# Autodesk Inventor assembly: Motor_25GA370-226x1-6V-21RPM
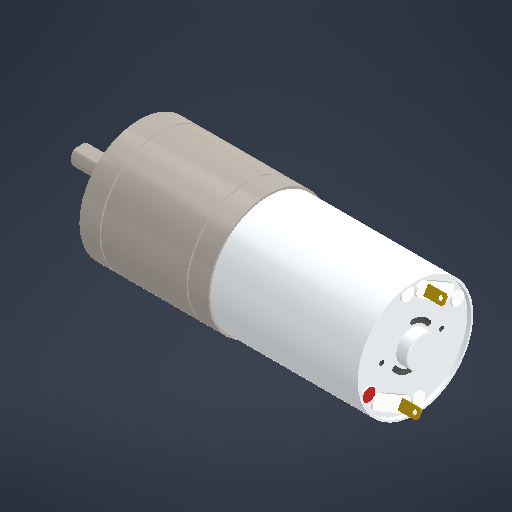
[picture p0: Inventor's stored thumbnail of the model, 512x512]
Saved by Autodesk Inventor 2026.1 (Build 301233000, 233)
## iProperties
Created: 2023-10-13
Part Number: Motor_25GA370-226x1-6V-21RPM
Description: STEP AP214
Document SubType Name: Assembly
Designer: pc
Sending System: SolidWorks 2022
Preprocessor: SwSTEP 2.0
Title: Motor_25GA370-226x1-6V-21RPM.STEP
Author: Wurs
Revision Number: ANY
## Documents named in this file (3)
- D:\momen\Eng.-ASU\Senior1\MCT Sys design\design\old design\Motor_25GA370-226x1-6V-21RPM.iam
- D:\momen\Eng.-ASU\Senior1\MCT Sys design\design\old design\Motor_25GA370-226x.ipt
- D:\momen\Eng.-ASU\Senior1\MCT Sys design\design\old design\pan cross head_am_B18.6.7M - M2.5 x 0.45 x 3 Type I Cross Recessed PHMS --3N.ipt
## Components (3 placed, 3 different names)
1. Motor_25GA370-226x_1 — Tangent:1
2. pan cross head_am_B18.6.7M - M2.5 x 0.45 x 3 Type I Cross Recessed PHMS --3N_2
3. pan cross head_am_B18.6.7M - M2.5 x 0.45 x 3 Type I Cross Recessed PHMS --3N_3
## Relationships (2: Angle 1, Tangent 1)
- Angle:1 (0 deg)
- Tangent:1: Motor_25GA370-226x_1
